# Autodesk Inventor assembly: MX-64AT_AR_sideL
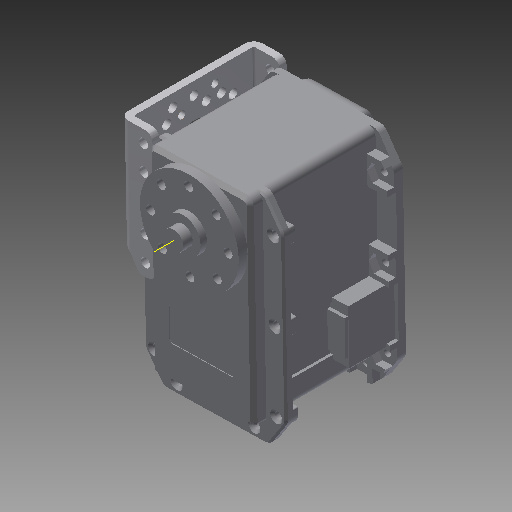
[picture p0: Inventor's stored thumbnail of the model, 512x512]
Saved by Autodesk Inventor 2018 (Build 220112000, 112)
## iProperties
Created: 2017-02-17
Part Number: MX-64AT_AR_sideL
Document SubType Name: Assembly
Designer: steve
Mass: 142.585 g
Surface Area: 190.405 cm^2
Volume: 74.8133 cm^3
Density: 1.90587 g/cm^3
Author: steve
## Documents named in this file (3)
- C:\Users\medrimonia\Dropbox\SigmaBan\SigmaBanV2.1\MX-64AT_AR_sideL.iam
- C:\Users\medrimonia\Dropbox\SigmaBan\SigmaBanV2.1\MX-64AT_AR.ipt
- C:\Users\medrimonia\Dropbox\SigmaBan\SigmaBanV2.1\FR05-S101.ipt
## Components (2 placed, 2 different names)
1. MX-64AT_AR:1 — Mate:1, Mate:2, Mate:3
2. FR05-S101:1 — Mate:1, Mate:2, Mate:3
## Relationships (3: Mate 3)
- Mate:1: MX-64AT_AR:1 ↔ FR05-S101:1
- Mate:2: MX-64AT_AR:1 ↔ FR05-S101:1
- Mate:3: MX-64AT_AR:1 ↔ FR05-S101:1
